# Autodesk Inventor assembly: Assembly3
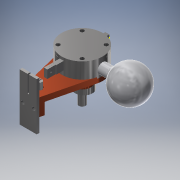
[picture p0: Inventor's stored thumbnail of the model, 180x180]
Saved by Autodesk Inventor 2018 (Build 220112000, 112)
## iProperties
Created: 2018-02-27
Part Number: Assembly3
Document SubType Name: Assembly
Designer: m234547
Author: m234547
## Documents named in this file (12)
- E:\ASSAMBLE\JIG SAW.iam
- E:\ASSAMBLE\Part1.ipt
- E:\ASSAMBLE\Part3.ipt
- E:\ASSAMBLE\Part4.ipt
- E:\ASSAMBLE\Part6.ipt
- E:\ASSAMBLE\Part9.ipt
- E:\ASSAMBLE\Part7.ipt
- E:\ASSAMBLE\Part8.ipt
- E:\ASSAMBLE\Part10.ipt
- E:\ASSAMBLE\Part5.ipt
- E:\ASSAMBLE\Part11.ipt
- E:\ASSAMBLE\Part2.ipt
## Components (11 placed, 11 different names)
1. Part1:1 — Mate:1, Flush:1, Mate:2, Mate:3, Mate:4, Mate:5, Insert:1, Mate:6, Insert:3, Mate:7, Mate:14, Mate:15, Flush:2, Mate:17
2. Part3:1 — Mate:3, Mate:4, Mate:5
3. Part4:1 — Insert:1, Mate:6, Insert:2
4. Part6:1 — Insert:2, Tangent:1, Mate:18
5. Part9:1 — Insert:3, Mate:7, Mate:8, Mate:9, Mate:12, Mate:13, Mate:16
6. Part7:1 — Mate:8, Mate:9, Tangent:1, Mate:10, Mate:11
7. Part8:1 — Mate:10, Mate:11
8. Part10:1 — Mate:12, Mate:13
9. Part5:1 — Mate:14, Mate:15
10. Part11:1 — Flush:2, Mate:16
11. Part2:1 — Mate:17, Mate:18
## Relationships (24: Mate 18, Insert 3, Flush 2, Tangent 1)
- Mate:1: Part1:1
- Flush:1: Part1:1
- Mate:2: Part1:1
- Mate:3: Part1:1 ↔ Part3:1
- Mate:4: Part1:1 ↔ Part3:1
- Mate:5: Part1:1 ↔ Part3:1
- Insert:1: Part1:1 ↔ Part4:1
- Mate:6: Part1:1 ↔ Part4:1
- Insert:2: Part4:1 ↔ Part6:1
- Insert:3: Part1:1 ↔ Part9:1
- Mate:7: Part1:1 ↔ Part9:1
- Mate:8: Part9:1 ↔ Part7:1
- Mate:9: Part9:1 ↔ Part7:1
- Tangent:1: Part6:1 ↔ Part7:1
- Mate:10: Part7:1 ↔ Part8:1
- Mate:11: Part7:1 ↔ Part8:1
- Mate:12: Part9:1 ↔ Part10:1
- Mate:13: Part9:1 ↔ Part10:1
- Mate:14: Part1:1 ↔ Part5:1
- Mate:15: Part1:1 ↔ Part5:1
- Flush:2 (30 mm): Part1:1 ↔ Part11:1
- Mate:16: Part9:1 ↔ Part11:1
- Mate:17: Part1:1 ↔ Part2:1
- Mate:18: Part6:1 ↔ Part2:1
